# Autodesk Inventor assembly: CamRightNCS
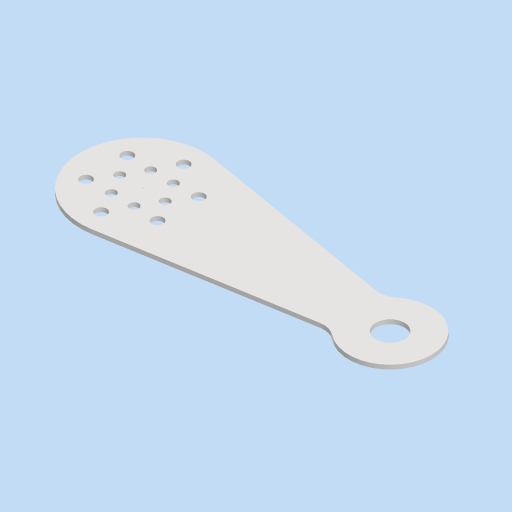
[picture p0: Inventor's stored thumbnail of the model, 512x512]
Saved by Autodesk Inventor 2023 (Build 270158000, 158)
## iProperties
Created: 2026-06-18
Part Number: CamRightNCS
Document SubType Name: Assembly
Designer: Nathann
Author: Nathann
## Documents named in this file (2)
- C:\Users\Nathann\ClawdDrive\Objet3D\RunningRobot\PartURDF\CamRightNCS.iam
- C:\Users\Nathann\ClawdDrive\Objet3D\RunningRobot\PartURDF\CamRight_Simplify_1.ipt
## Components (1 placed, 1 different names)
1. CamRight_Simplify_1:1 — Mate:1, Flush:1, Angle:1
## Relationships (5: Mate 3, Flush 1, Angle 1)
- Mate:1: CamRight_Simplify_1:1
- Mate:2
- Mate:3
- Flush:1: CamRight_Simplify_1:1
- Angle:1 (0 deg): CamRight_Simplify_1:1
